# Autodesk Inventor assembly: Assembly
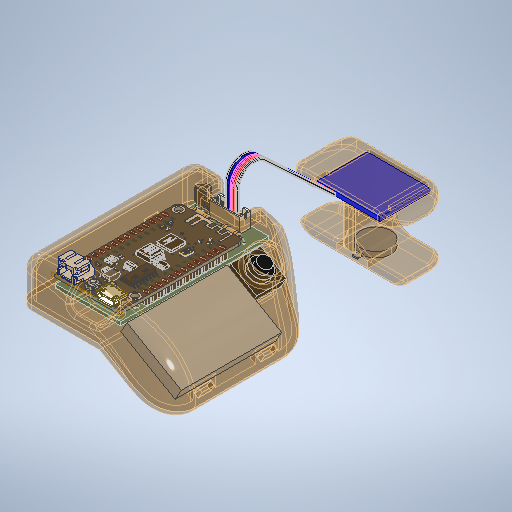
[picture p0: Inventor's stored thumbnail of the model, 512x512]
Saved by Autodesk Inventor 2025.2 (Build 292293000, 293)
## iProperties
Created: 2025-08-11
Part Number: Assembly
Document SubType Name: Assembly
Designer: naka6
Author: naka6
## Documents named in this file (11)
- C:\Users\naka6\OneDrive\ドキュメント\ARSS\3DCAD\Assembly.iam
- C:\Users\naka6\OneDrive\ドキュメント\ARSS\3DCAD\Cuicuit\Cuicuit.iam
- C:\Users\naka6\OneDrive\ドキュメント\ARSS\3DCAD\lolin32-lite-1.snapshot.18\Lolin32 Lite - Male Headers\Lolin32 Lite - Male Headers.iam
- C:\Users\naka6\OneDrive\ドキュメント\ARSS\3DCAD\switch.ipt
- C:\Users\naka6\OneDrive\ドキュメント\ARSS\3DCAD\batery.ipt
- C:\Users\naka6\OneDrive\ドキュメント\ARSS\3DCAD\case.ipt
- C:\Users\naka6\OneDrive\ドキュメント\ARSS\3DCAD\caber.ipt
- C:\Users\naka6\OneDrive\ドキュメント\ARSS\3DCAD\BNO055.ipt
- C:\Users\naka6\OneDrive\ドキュメント\ARSS\3DCAD\ring_base.ipt
- C:\Users\naka6\OneDrive\ドキュメント\ARSS\3DCAD\motor.ipt
- C:\Users\naka6\OneDrive\ドキュメント\ARSS\3DCAD\cable.ipt
## Components (14 placed, 10 different names)
1. Cuicuit:1 [sub-assembly] — フラッシュ:1, フラッシュ:2, メイト:1, メイト:2, 角度:1, フラッシュ:3, メイト:7, メイト:8, フラッシュ:7, フラッシュ:11, フラッシュ:12, フラッシュ:13
2. Lolin32 Lite - Male Headers:1 [sub-assembly] — フラッシュ:1, フラッシュ:2, メイト:1, フラッシュ:10, フラッシュ:15
3. switch:1 — メイト:5, メイト:6, フラッシュ:8, フラッシュ:9, フラッシュ:14
4. batery:1 — メイト:3, メイト:4, フラッシュ:7
5. case:1 — メイト:3, メイト:4, メイト:5, メイト:6, フラッシュ:3, メイト:7, メイト:8, フラッシュ:4, フラッシュ:5, フラッシュ:6, フラッシュ:14
6. caber:1 — フラッシュ:4, フラッシュ:5, フラッシュ:6, フラッシュ:8, フラッシュ:9, フラッシュ:10, フラッシュ:11, フラッシュ:12, フラッシュ:13, フラッシュ:15
7. BNO055:1 — 角度:2, 角度:3, メイト:10, メイト:11, メイト:12
8. ring_base:1 — 角度:3, メイト:10, メイト:11, メイト:12, 正接:1, メイト:13
9. motor:1 — 角度:4, 正接:1, メイト:13
10. cable:1
11. cable:2
12. cable:3
13. cable:4
14. cable:6
## Relationships (32: Flush 15, Mate 12, Angle 4, Tangent 1)
- フラッシュ:1 [Flush] (0.1 mm): Cuicuit:1 ↔ Lolin32 Lite - Male Headers:1
- フラッシュ:2 [Flush] (-0.334 mm): Cuicuit:1 ↔ Lolin32 Lite - Male Headers:1
- メイト:1 [Mate]: Cuicuit:1 ↔ Lolin32 Lite - Male Headers:1
- メイト:2 [Mate]: Cuicuit:1
- 角度:1 [Angle] (0 deg): Cuicuit:1
- メイト:3 [Mate]: batery:1 ↔ case:1
- メイト:4 [Mate]: batery:1 ↔ case:1
- メイト:5 [Mate]: switch:1 ↔ case:1
- メイト:6 [Mate]: switch:1 ↔ case:1
- フラッシュ:3 [Flush] (2.5 mm): Cuicuit:1 ↔ case:1
- メイト:7 [Mate] (2 mm): Cuicuit:1 ↔ case:1
- メイト:8 [Mate]: Cuicuit:1 ↔ case:1
- フラッシュ:4 [Flush]: case:1 ↔ caber:1
- フラッシュ:5 [Flush]: case:1 ↔ caber:1
- フラッシュ:6 [Flush]: case:1 ↔ caber:1
- フラッシュ:7 [Flush]: Cuicuit:1 ↔ batery:1
- フラッシュ:8 [Flush]: switch:1 ↔ caber:1
- フラッシュ:9 [Flush] (-1 mm): switch:1 ↔ caber:1
- フラッシュ:10 [Flush]: Lolin32 Lite - Male Headers:1 ↔ caber:1
- フラッシュ:11 [Flush]: Cuicuit:1 ↔ caber:1
- フラッシュ:12 [Flush]: Cuicuit:1 ↔ caber:1
- フラッシュ:13 [Flush]: Cuicuit:1 ↔ caber:1
- フラッシュ:14 [Flush] (8 mm): switch:1 ↔ case:1
- フラッシュ:15 [Flush]: Lolin32 Lite - Male Headers:1 ↔ caber:1
- 角度:2 [Angle] (0 deg): BNO055:1
- 角度:3 [Angle] (0 deg): BNO055:1 ↔ ring_base:1
- メイト:10 [Mate]: BNO055:1 ↔ ring_base:1
- メイト:11 [Mate]: BNO055:1 ↔ ring_base:1
- メイト:12 [Mate] (0.25 mm): BNO055:1 ↔ ring_base:1
- 角度:4 [Angle] (0 deg): motor:1
- 正接:1 [Tangent]: ring_base:1 ↔ motor:1
- メイト:13 [Mate]: ring_base:1 ↔ motor:1
